# Autodesk Inventor assembly: ElectronicsBatteryAssembly
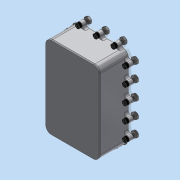
[picture p0: Inventor's stored thumbnail of the model, 180x180]
Saved by Autodesk Inventor 2017 (Build 210142000, 142)
## iProperties
Created: 2018-02-14
Part Number: ElectronicsBatteryAssembly
Document SubType Name: Assembly
Designer: Derek Wider
Author: Derek Wider
## Documents named in this file (12)
- G:\Projects\Submarine\Submarine-project\CAD\common\ElectronicsBatteryAssembly.iam
- G:\Projects\Submarine\Submarine-project\CAD\common\ElectronicsBatteryNoConnector.ipt
- G:\Projects\Submarine\Submarine-project\CAD\common\Connectors\XT60\XT60 Connector Female Connector.iam
- G:\Projects\Submarine\Submarine-project\CAD\fore\BatteryCaseSide1.ipt
- G:\Projects\Submarine\Submarine-project\CAD\fore\BatteryCaseSide2.ipt
- G:\Projects\Submarine\Submarine-project\CAD\fore\BatteryCaseORing.ipt
- G:\Projects\Submarine\Submarine-project\CAD\fore\BatteryCaseSide3.ipt
- G:\Projects\Submarine\Submarine-project\CAD\common\ThreadedRod_Nuts_Bolts\Bolt_SocketHead_Hex_Thread_5_40_7_16length.ipt
- G:\Projects\Submarine\Submarine-project\CAD\common\ThreadedRod_Nuts_Bolts\NarrowHexNutThread_5_40.ipt
- G:\Projects\Submarine\Submarine-project\CAD\fore\BatteryCaseBlackWire.ipt
- G:\Projects\Submarine\Submarine-project\CAD\fore\BatteryCaseRedWire.ipt
- G:\Projects\Submarine\Submarine-project\CAD\common\Connectors\XT60\XT60 Connector Male Connector.iam
## Components (41 placed, 11 different names)
1. ElectronicsBatteryNoConnector:1 — Mate:1, Mate:2, Angle:1, Mate:6, Mate:7, Mate:8
2. XT60 Connector Female Connector:1 [sub-assembly] — Mate:1, Mate:2, Angle:1
3. BatteryCaseSide1:1 — Tangent:1, Tangent:2, Tangent:3, Tangent:4, Mate:5, Flush:1, Flush:2, Mate:7, Mate:8, Mate:9, Flush:3, Flush:4, Mate:10, Mate:11, Mate:12, Mate:13, Mate:18, Mate:19, Angle:2, Mate:23
4. BatteryCaseSide2:1 — Mate:9, Flush:3, Flush:4, Mate:14, Mate:17
5. BatteryCaseORing:1 — Tangent:1, Tangent:2, Tangent:3, Tangent:4
6. BatteryCaseSide3:1 — Mate:5, Flush:1, Flush:2, Mate:6
7. BatteryCaseBlackWire:1 — Mate:18, Mate:22
8. BatteryCaseRedWire:1 — Mate:19, Mate:20, Mate:21
9. XT60 Connector Male Connector:1 [sub-assembly] — Mate:20, Mate:21, Mate:22, Angle:2, Mate:23
10. Bolt_SocketHead_Hex_Thread_5_40_7_16length:1 — Mate:10, Mate:11
11. Bolt_SocketHead_Hex_Thread_5_40_7_16length:2 — Mate:15
12. Bolt_SocketHead_Hex_Thread_5_40_7_16length:3
13. Bolt_SocketHead_Hex_Thread_5_40_7_16length:4
14. Bolt_SocketHead_Hex_Thread_5_40_7_16length:5
15. Bolt_SocketHead_Hex_Thread_5_40_7_16length:6
16. Bolt_SocketHead_Hex_Thread_5_40_7_16length:7
17. Bolt_SocketHead_Hex_Thread_5_40_7_16length:8
18. Bolt_SocketHead_Hex_Thread_5_40_7_16length:9
19. Bolt_SocketHead_Hex_Thread_5_40_7_16length:10
20. Bolt_SocketHead_Hex_Thread_5_40_7_16length:11 — Mate:12, Mate:13
21. Bolt_SocketHead_Hex_Thread_5_40_7_16length:12
22. Bolt_SocketHead_Hex_Thread_5_40_7_16length:13
23. Bolt_SocketHead_Hex_Thread_5_40_7_16length:14
24. Bolt_SocketHead_Hex_Thread_5_40_7_16length:15 — Mate:16
25. Bolt_SocketHead_Hex_Thread_5_40_7_16length:16
26. NarrowHexNutThread_5_40:1 — Mate:14, Mate:15
27. NarrowHexNutThread_5_40:2
28. NarrowHexNutThread_5_40:3
29. NarrowHexNutThread_5_40:4
30. NarrowHexNutThread_5_40:5
31. NarrowHexNutThread_5_40:6
32. NarrowHexNutThread_5_40:7
33. NarrowHexNutThread_5_40:8
34. NarrowHexNutThread_5_40:9
35. NarrowHexNutThread_5_40:10
36. NarrowHexNutThread_5_40:11 — Mate:16, Mate:17
37. NarrowHexNutThread_5_40:12
38. NarrowHexNutThread_5_40:13
39. NarrowHexNutThread_5_40:14
40. NarrowHexNutThread_5_40:15
41. NarrowHexNutThread_5_40:16
## Component patterns: (10 elements, first: Bolt_SocketHead_Hex_Thread_5_40_7_16length:1), (6 elements, first: Bolt_SocketHead_Hex_Thread_5_40_7_16length:11), (10 elements, first: NarrowHexNutThread_5_40:1), (6 elements, first: NarrowHexNutThread_5_40:11)
## Relationships (31: Mate 21, Tangent 4, Flush 4, Angle 2)
- Mate:1: ElectronicsBatteryNoConnector:1 ↔ XT60 Connector Female Connector:1
- Mate:2: ElectronicsBatteryNoConnector:1 ↔ XT60 Connector Female Connector:1
- Angle:1 (0 deg): ElectronicsBatteryNoConnector:1 ↔ XT60 Connector Female Connector:1
- Tangent:1: BatteryCaseSide1:1 ↔ BatteryCaseORing:1
- Tangent:2: BatteryCaseSide1:1 ↔ BatteryCaseORing:1
- Tangent:3 (1.27 mm): BatteryCaseSide1:1 ↔ BatteryCaseORing:1
- Tangent:4 (1.27 mm): BatteryCaseSide1:1 ↔ BatteryCaseORing:1
- Mate:5: BatteryCaseSide1:1 ↔ BatteryCaseSide3:1
- Flush:1: BatteryCaseSide1:1 ↔ BatteryCaseSide3:1
- Flush:2: BatteryCaseSide1:1 ↔ BatteryCaseSide3:1
- Mate:6: ElectronicsBatteryNoConnector:1 ↔ BatteryCaseSide3:1
- Mate:7 (6.35 mm): ElectronicsBatteryNoConnector:1 ↔ BatteryCaseSide1:1
- Mate:8 (6.35 mm): ElectronicsBatteryNoConnector:1 ↔ BatteryCaseSide1:1
- Mate:9: BatteryCaseSide1:1 ↔ BatteryCaseSide2:1
- Flush:3: BatteryCaseSide1:1 ↔ BatteryCaseSide2:1
- Flush:4: BatteryCaseSide1:1 ↔ BatteryCaseSide2:1
- Mate:10: BatteryCaseSide1:1 ↔ Bolt_SocketHead_Hex_Thread_5_40_7_16length:1
- Mate:11: BatteryCaseSide1:1 ↔ Bolt_SocketHead_Hex_Thread_5_40_7_16length:1
- Mate:12: BatteryCaseSide1:1 ↔ Bolt_SocketHead_Hex_Thread_5_40_7_16length:11
- Mate:13: BatteryCaseSide1:1 ↔ Bolt_SocketHead_Hex_Thread_5_40_7_16length:11
- Mate:14: BatteryCaseSide2:1 ↔ NarrowHexNutThread_5_40:1
- Mate:15: Bolt_SocketHead_Hex_Thread_5_40_7_16length:2 ↔ NarrowHexNutThread_5_40:1
- Mate:16: Bolt_SocketHead_Hex_Thread_5_40_7_16length:15 ↔ NarrowHexNutThread_5_40:11
- Mate:17: BatteryCaseSide2:1 ↔ NarrowHexNutThread_5_40:11
- Mate:18: BatteryCaseSide1:1 ↔ BatteryCaseBlackWire:1
- Mate:19: BatteryCaseSide1:1 ↔ BatteryCaseRedWire:1
- Mate:20: BatteryCaseRedWire:1 ↔ XT60 Connector Male Connector:1
- Mate:21: BatteryCaseRedWire:1 ↔ XT60 Connector Male Connector:1
- Mate:22: BatteryCaseBlackWire:1 ↔ XT60 Connector Male Connector:1
- Angle:2 (0 deg): BatteryCaseSide1:1 ↔ XT60 Connector Male Connector:1
- Mate:23 (9.525 mm): BatteryCaseSide1:1 ↔ XT60 Connector Male Connector:1
